# Autodesk Inventor assembly: Red Alliance Arm
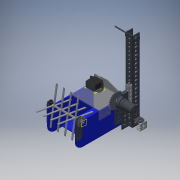
[picture p0: Inventor's stored thumbnail of the model, 180x180]
Saved by Autodesk Inventor 2016 (Build 200138000, 138)
## iProperties
Created: 2015-12-20
Part Number: Red Alliance Arm
Document SubType Name: Assembly
Designer: tbloo
Author: tbloo
## Documents named in this file (13)
- C:\Users\TimB\Documents\GitHub\phi_robotics\3d-models\FTC_Tetrix_KOP_Block_Party\Tim Bloot Designs\JAr JaR Bot\Blue Alliance Arm.iam
- C:\Users\TimB\Documents\GitHub\phi_robotics\3d-models\FTC_Tetrix_KOP_Block_Party\Tetrix_Kit_FTC\Autodesk Inventor Files\tetrix_axle.ipt
- C:\Users\TimB\Documents\GitHub\phi_robotics\3d-models\FTC_Tetrix_KOP_Block_Party\Tetrix_Kit_FTC\Autodesk Inventor Files\tetrix_axle_lock.iam
- C:\Users\TimB\Documents\GitHub\phi_robotics\3d-models\FTC_Tetrix_KOP_Block_Party\Tim Bloot Designs\JAr JaR Bot\cube channel short.ipt
- C:\Users\TimB\Documents\GitHub\phi_robotics\3d-models\FTC_Tetrix_KOP_Block_Party\Tetrix_Kit_FTC\Autodesk Inventor Files\tetrix_motor_mount-old.ipt
- C:\Users\TimB\Documents\GitHub\phi_robotics\3d-models\FTC_Tetrix_KOP_Block_Party\Tetrix_Kit_FTC\Autodesk Inventor Files\tetrix_motor.iam
- C:\Users\TimB\Documents\GitHub\phi_robotics\3d-models\FTC_Tetrix_KOP_Block_Party\Tetrix_Kit_FTC\Autodesk Inventor Files\tetrix_maxle_lock.iam
- C:\Users\TimB\Documents\GitHub\phi_robotics\3d-models\FTC_Tetrix_KOP_Block_Party\Tetrix_Kit_FTC\Autodesk Inventor Files\tetrix_chain_gear-32t.ipt
- C:\Users\TimB\Documents\GitHub\phi_robotics\3d-models\FTC_Tetrix_KOP_Block_Party\Tetrix_Kit_FTC\Autodesk Inventor Files\tetrix_c_channel-2.ipt
- C:\Users\TimB\Documents\GitHub\phi_robotics\3d-models\FTC_Tetrix_KOP_Block_Party\Tim Bloot Designs\JAr JaR Bot\Blue Alliance Bucket.iam
- C:\Users\TimB\Documents\GitHub\phi_robotics\3d-models\FTC_Tetrix_KOP_Block_Party\Tetrix_Kit_FTC\Autodesk Inventor Files\tetrix_c_channel-round.ipt
- C:\Users\TimB\Documents\GitHub\phi_robotics\3d-models\FTC_Tetrix_KOP_Block_Party\Tetrix_Kit_FTC\Autodesk Inventor Files\tetrix_Lbracket-round.ipt
- C:\Users\TimB\Documents\GitHub\phi_robotics\3d-models\FTC_Tetrix_KOP_Block_Party\Tim Bloot Designs\JAr JaR Bot\cut c channel.ipt
## Components (13 placed, 12 different names)
1. tetrix_axle:1 — Rigid:5
2. tetrix_axle_lock:1 [sub-assembly] — Rigid:5, Rigid:18
3. tetrix_axle_lock:2 [sub-assembly] — Rigid:14
4. cube channel short:1 — Rigid:10, Rigid:17
5. tetrix_motor_mount-old:1 — Rigid:10, Rotational:1
6. tetrix_motor:1 [sub-assembly] — Rigid:9, Rotational:1
7. tetrix_maxle_lock:1 [sub-assembly] — Rigid:9
8. tetrix_chain_gear-32t:1
9. tetrix_c_channel-2:1 — Mate:1, Flush:1, Flush:2, Rigid:16
10. Blue Alliance Bucket:1 [sub-assembly] — Mate:1, Flush:1, Flush:2
11. tetrix_c_channel-round:1 — Rigid:13
12. tetrix_Lbracket-round:1 — Rigid:13, Rigid:15
13. cut c channel:1 — Rigid:14, Rigid:15, Rigid:16, Rigid:17, Rigid:18
## Relationships (14: WeldJoint 10, Flush 2, RevoluteJoint 1, Mate 1)
- Rigid:5 [WeldJoint]: tetrix_axle:1 ↔ tetrix_axle_lock:1
- [WeldJoint]: tetrix_maxle_lock:1 ↔ tetrix_chain_gear-32t:1
- Rigid:9 [WeldJoint] (-7 mm): tetrix_motor:1 ↔ tetrix_maxle_lock:1
- Rigid:10 [WeldJoint]: cube channel short:1 ↔ tetrix_motor_mount-old:1
- Rotational:1 [RevoluteJoint]: tetrix_motor_mount-old:1 ↔ tetrix_motor:1
- Mate:1: tetrix_c_channel-2:1 ↔ Blue Alliance Bucket:1
- Flush:1: tetrix_c_channel-2:1 ↔ Blue Alliance Bucket:1
- Flush:2 (10 mm): tetrix_c_channel-2:1 ↔ Blue Alliance Bucket:1
- Rigid:13 [WeldJoint]: tetrix_c_channel-round:1 ↔ tetrix_Lbracket-round:1
- Rigid:14 [WeldJoint]: tetrix_axle_lock:2 ↔ cut c channel:1
- Rigid:15 [WeldJoint]: tetrix_Lbracket-round:1 ↔ cut c channel:1
- Rigid:16 [WeldJoint]: tetrix_c_channel-2:1 ↔ cut c channel:1
- Rigid:17 [WeldJoint]: cube channel short:1 ↔ cut c channel:1
- Rigid:18 [WeldJoint]: tetrix_axle_lock:1 ↔ cut c channel:1
## Named parameters: d13_d12 = 0 mm
